# Autodesk Inventor assembly: Chessboard Bottom
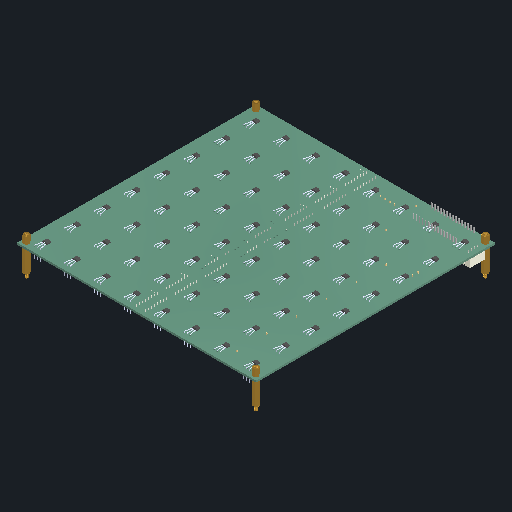
[picture p0: Inventor's stored thumbnail of the model, 512x512]
Saved by Autodesk Inventor 2026 (Build 300175000, 175)
## iProperties
Created: 2025-04-19
Part Number: Chessboard Bottom
Document SubType Name: Assembly
Designer: ckyiu
Author: ckyiu
## Documents named in this file (4)
- F:\Chessboard-Design\Design\Core\Chessboard Bottom.iam
- F:\Chessboard-Design\Design\Core\PCBs\Parts\Chessboard Hardware Model.iam
- F:\Chessboard-Design\Design\Hardware\M2.5\Standoffs\M-F\(20mm) 98952A117_Aluminum Male-Female Threaded Hex Standoff.ipt
- F:\Chessboard-Design\Design\Hardware\M2.5\Standoffs\M-F\(6mm) 98952A103_Aluminum Male-Female Threaded Hex Standoff.ipt
## Components (9 placed, 3 different names)
1. Chessboard Hardware Model:1 [sub-assembly] — Insert:1, Insert:2, Insert:3, Insert:4, Insert:5, Insert:6, Insert:7, Insert:8
2. (6mm) 98952A103_Aluminum Male-Female Threaded Hex Standoff:1 — Insert:1
3. (6mm) 98952A103_Aluminum Male-Female Threaded Hex Standoff:2 — Insert:2
4. (6mm) 98952A103_Aluminum Male-Female Threaded Hex Standoff:3 — Insert:3
5. (6mm) 98952A103_Aluminum Male-Female Threaded Hex Standoff:4 — Insert:4
6. (20mm) 98952A117_Aluminum Male-Female Threaded Hex Standoff:1 — Insert:5
7. (20mm) 98952A117_Aluminum Male-Female Threaded Hex Standoff:2 — Insert:6
8. (20mm) 98952A117_Aluminum Male-Female Threaded Hex Standoff:3 — Insert:8
9. (20mm) 98952A117_Aluminum Male-Female Threaded Hex Standoff:4 — Insert:7
## Relationships (8: Insert 8)
- Insert:1: Chessboard Hardware Model:1 ↔ (6mm) 98952A103_Aluminum Male-Female Threaded Hex Standoff:1
- Insert:2: Chessboard Hardware Model:1 ↔ (6mm) 98952A103_Aluminum Male-Female Threaded Hex Standoff:2
- Insert:3: Chessboard Hardware Model:1 ↔ (6mm) 98952A103_Aluminum Male-Female Threaded Hex Standoff:3
- Insert:4: Chessboard Hardware Model:1 ↔ (6mm) 98952A103_Aluminum Male-Female Threaded Hex Standoff:4
- Insert:5: Chessboard Hardware Model:1 ↔ (20mm) 98952A117_Aluminum Male-Female Threaded Hex Standoff:1
- Insert:6: Chessboard Hardware Model:1 ↔ (20mm) 98952A117_Aluminum Male-Female Threaded Hex Standoff:2
- Insert:7: Chessboard Hardware Model:1 ↔ (20mm) 98952A117_Aluminum Male-Female Threaded Hex Standoff:4
- Insert:8: Chessboard Hardware Model:1 ↔ (20mm) 98952A117_Aluminum Male-Female Threaded Hex Standoff:3
